# Autodesk Inventor assembly: PlanetaryGear
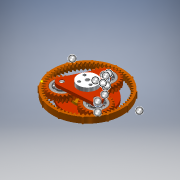
[picture p0: Inventor's stored thumbnail of the model, 180x180]
Saved by Autodesk Inventor 2018.3 (Build 223284000, 284)
## iProperties
Created: 2018-07-08
Part Number: PlanetaryGear
Material: Generisch
Document SubType Name: Assembly
Designer: JochenAlt
Author: JochenAlt
## Documents named in this file (11)
- D:\Projects\FlowerPot\CAD\PlanetaryGear\PlanetaryGear.iam
- D:\Projects\FlowerPot\CAD\PlanetaryGear\Konstruktions-Assistent\Stirnzahnrad21.ipt
- D:\Projects\FlowerPot\CAD\PlanetaryGear\Konstruktions-Assistent\Stirnzahnrad23.ipt
- D:\Projects\FlowerPot\CAD\PlanetaryGear\PlanetaryHolder.ipt
- D:\Projects\FlowerPot\CAD\PlanetaryGear\PlanetaryHolderTop.ipt
- D:\Projects\FlowerPot\CAD\Mounting Hub.ipt
- D:\Projects\FlowerPot\CAD\PlanetaryGear\PlanetaryHolderBottom.ipt
- D:\Projects\FlowerPot\CAD\PlanetaryGear\PlanetaryGearConstr\Konstruktions-Assistent\Stirnzahnrad12.ipt
- C:\Users\JochenAlt\Documents\Inventor\Content Center Files\R2018\de-DE\DIN BEARING(1)\DIN 625 SKF - SKF 626.ipt
- C:\Users\JochenAlt\Documents\Inventor\Content Center Files\R2018\de-DE\DIN 912\DIN 912 - M2 x 0,4 x 12 x 11.ipt
- C:\Users\JochenAlt\Documents\Inventor\Content Center Files\R2018\de-DE\DIN 934\DIN 934 - M2 x 0,4.ipt
## Components (18 placed, 9 different names)
1. Stirnzahnrad2:1 — Fluchtend:1, Passend:13
2. Stirnzahnrad2:2 — Fluchtend:1, Fluchtend:4, Fluchtend:5, Passend:16, Drehung:9, Passend:32
3. Stirnzahnrad2:3 — Fluchtend:3, Passend:18, Passend:29, Drehung:6, Passend:31
4. Stirnzahnrad2:4 — Fluchtend:2, Fluchtend:6, Passend:17, Drehung:7, Passend:34
5. PlanetaryHolder:1
6. PlanetaryHolderTop:1 — Passend:1, Passend:2, Passend:26, Passend:27, Passend:28, Passend:29, Passend:42, Passend:44, Passend:46
7. Mounting Hub:1 — Passend:1, Passend:2
8. PlanetaryHolderBottom:1 — Passend:15, Passend:16, Passend:17, Passend:18, Passend:23, Passend:25, Passend:26, Passend:27, Passend:28, Drehung:5, Passend:33, Passend:35, Passend:36, Passend:37, Passend:38, Passend:39, Passend:40
9. Stirnzahnrad1:1 — Fluchtend:2, Passend:14, Fluchtend:3, Fluchtend:4, Fluchtend:5, Fluchtend:6, Drehung:5, Drehung:6, Drehung:7, Drehung:9
10. DIN 625 SKF SKF 626:1 — Passend:23, Passend:32
11. DIN 625 SKF SKF 626:2 — Passend:33, Passend:34
12. DIN 625 SKF SKF 626:3 — Passend:25, Passend:31
13. DIN 912 - ersetzt durch DIN EN ISO 4762 M2 x 12:1 — Passend:35, Passend:36, Passend:45
14. DIN 912 - ersetzt durch DIN EN ISO 4762 M2 x 12:2 — Passend:37, Passend:38, Passend:43
15. DIN 912 - ersetzt durch DIN EN ISO 4762 M2 x 12:3 — Passend:39, Passend:40, Passend:41
16. DIN 934 - ersetzt durch DIN EN 24032/28673/28674 M2:1 — Passend:41, Passend:42
17. DIN 934 - ersetzt durch DIN EN 24032/28673/28674 M2:2 — Passend:43, Passend:44
18. DIN 934 - ersetzt durch DIN EN 24032/28673/28674 M2:3 — Passend:45, Passend:46
## Relationships (40: Mate 30, Flush 6, RelateRotation 4)
- Passend:1 [Mate]: PlanetaryHolderTop:1 ↔ Mounting Hub:1
- Passend:2 [Mate]: PlanetaryHolderTop:1 ↔ Mounting Hub:1
- Fluchtend:1 [Flush]: Stirnzahnrad2:1 ↔ Stirnzahnrad2:2
- Fluchtend:2 [Flush]: Stirnzahnrad2:4 ↔ Stirnzahnrad1:1
- Passend:13 [Mate]: Stirnzahnrad2:1
- Passend:14 [Mate]: Stirnzahnrad1:1
- Passend:15 [Mate]: PlanetaryHolderBottom:1
- Fluchtend:3 [Flush]: Stirnzahnrad2:3 ↔ Stirnzahnrad1:1
- Fluchtend:4 [Flush]: Stirnzahnrad2:2 ↔ Stirnzahnrad1:1
- Fluchtend:5 [Flush]: Stirnzahnrad2:2 ↔ Stirnzahnrad1:1
- Fluchtend:6 [Flush]: Stirnzahnrad2:4 ↔ Stirnzahnrad1:1
- Passend:16 [Mate]: Stirnzahnrad2:2 ↔ PlanetaryHolderBottom:1
- Passend:17 [Mate]: Stirnzahnrad2:4 ↔ PlanetaryHolderBottom:1
- Passend:18 [Mate]: Stirnzahnrad2:3 ↔ PlanetaryHolderBottom:1
- Passend:23 [Mate]: PlanetaryHolderBottom:1 ↔ DIN 625 SKF SKF 626:1
- Passend:25 [Mate]: PlanetaryHolderBottom:1 ↔ DIN 625 SKF SKF 626:3
- Passend:26 [Mate]: PlanetaryHolderTop:1 ↔ PlanetaryHolderBottom:1
- Passend:27 [Mate]: PlanetaryHolderTop:1 ↔ PlanetaryHolderBottom:1
- Passend:28 [Mate]: PlanetaryHolderTop:1 ↔ PlanetaryHolderBottom:1
- Drehung:5 [RelateRotation] (-0.2 ul): PlanetaryHolderBottom:1 ↔ Stirnzahnrad1:1
- Passend:29 [Mate] (1 mm): Stirnzahnrad2:3 ↔ PlanetaryHolderTop:1
- Drehung:6 [RelateRotation] (-0.29 ul): Stirnzahnrad2:3 ↔ Stirnzahnrad1:1
- Drehung:7 [RelateRotation] (-0.2884 ul): Stirnzahnrad2:4 ↔ Stirnzahnrad1:1
- Drehung:9 [RelateRotation] (0.29 ul): Stirnzahnrad2:2 ↔ Stirnzahnrad1:1
- Passend:31 [Mate]: Stirnzahnrad2:3 ↔ DIN 625 SKF SKF 626:3
- Passend:32 [Mate]: Stirnzahnrad2:2 ↔ DIN 625 SKF SKF 626:1
- Passend:33 [Mate]: PlanetaryHolderBottom:1 ↔ DIN 625 SKF SKF 626:2
- Passend:34 [Mate]: Stirnzahnrad2:4 ↔ DIN 625 SKF SKF 626:2
- Passend:35 [Mate]: PlanetaryHolderBottom:1 ↔ DIN 912 - ersetzt durch DIN EN ISO 4762 M2 x 12:1
- Passend:36 [Mate]: PlanetaryHolderBottom:1 ↔ DIN 912 - ersetzt durch DIN EN ISO 4762 M2 x 12:1
- Passend:37 [Mate]: PlanetaryHolderBottom:1 ↔ DIN 912 - ersetzt durch DIN EN ISO 4762 M2 x 12:2
- Passend:38 [Mate]: PlanetaryHolderBottom:1 ↔ DIN 912 - ersetzt durch DIN EN ISO 4762 M2 x 12:2
- Passend:39 [Mate]: PlanetaryHolderBottom:1 ↔ DIN 912 - ersetzt durch DIN EN ISO 4762 M2 x 12:3
- Passend:40 [Mate]: PlanetaryHolderBottom:1 ↔ DIN 912 - ersetzt durch DIN EN ISO 4762 M2 x 12:3
- Passend:41 [Mate]: DIN 912 - ersetzt durch DIN EN ISO 4762 M2 x 12:3 ↔ DIN 934 - ersetzt durch DIN EN 24032/28673/28674 M2:1
- Passend:42 [Mate]: PlanetaryHolderTop:1 ↔ DIN 934 - ersetzt durch DIN EN 24032/28673/28674 M2:1
- Passend:43 [Mate]: DIN 912 - ersetzt durch DIN EN ISO 4762 M2 x 12:2 ↔ DIN 934 - ersetzt durch DIN EN 24032/28673/28674 M2:2
- Passend:44 [Mate]: PlanetaryHolderTop:1 ↔ DIN 934 - ersetzt durch DIN EN 24032/28673/28674 M2:2
- Passend:45 [Mate]: DIN 912 - ersetzt durch DIN EN ISO 4762 M2 x 12:1 ↔ DIN 934 - ersetzt durch DIN EN 24032/28673/28674 M2:3
- Passend:46 [Mate]: PlanetaryHolderTop:1 ↔ DIN 934 - ersetzt durch DIN EN 24032/28673/28674 M2:3
